# Autodesk Inventor assembly: 25203-02
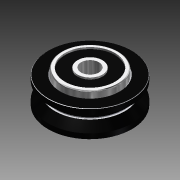
[picture p0: Inventor's stored thumbnail of the model, 180x180]
Saved by Autodesk Inventor 2014 (Build 180170000, 170)
## iProperties
Created: 2012-01-16
Part Number: 25203-02
Document SubType Name: Assembly
Designer: ERF
Description: Dual Bearing V Wheel Kit (assembly)
Mass: 3.05191 g
Surface Area: 39.551 cm^2
Volume: 2.4421 cm^3
Density: 1.24971 g/cm^3
Vendor: custom
Stock Number: B30037_ASM
Project: Shapeoko
User Status: F
Author: ERF
Subject: Motion
Title: V-Wheel Assembly
## Documents named in this file (4)
- C:\Users\Edward\Documents\GitHub\Shapeoko_2\Autodesk_Inventor_Project\25203-02.iam
- C:\Users\Edward\Documents\GitHub\Shapeoko_2\Autodesk_Inventor_Project\25202-01.ipt
- C:\Users\Edward\Documents\GitHub\Shapeoko_2\Autodesk_Inventor_Project\25196-01.ipt
- C:\Users\Edward\Documents\GitHub\Shapeoko_2\Autodesk_Inventor_Project\25201-01.ipt
## Components (4 placed, 3 different names)
1. 25202-01:1 — Insert:1, Insert:3
2. 25196-01:1 — Insert:3
3. 25201-01:1 — Insert:4
4. 25196-01:2 — Insert:1, Insert:4
## Relationships (3: Insert 3)
- Insert:1: 25202-01:1 ↔ 25196-01:2
- Insert:3: 25202-01:1 ↔ 25196-01:1
- Insert:4: 25201-01:1 ↔ 25196-01:2
